# Autodesk Inventor assembly: bodyAssembly
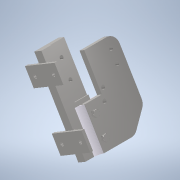
[picture p0: Inventor's stored thumbnail of the model, 180x180]
Saved by Autodesk Inventor 2020.3 (Build 243373000, 373)
## iProperties
Created: 2021-06-21
Part Number: bodyAssembly
Document SubType Name: Weldment
Designer: 0x6f736f646f
Weld Material: Welded Aluminum-6061
Author: 0x6f736f646f
## Documents named in this file (7)
- C:\Users\Public\D\Desktop\Trash\Manufacturing-Technology-1-Project\bodyAssembly.iam
- C:\Users\Public\D\Desktop\Trash\Manufacturing-Technology-1-Project\bodybottompart.ipt
- C:\Users\Public\D\Desktop\Trash\Manufacturing-Technology-1-Project\bodystandoff.ipt
- C:\Users\Public\D\Desktop\Trash\Manufacturing-Technology-1-Project\bodytoppart.ipt
- C:\Users\0x6f736f646f\OneDrive\Documents\Inventor\Content Center Files\R2020\en-US\BS EN ISO 8765\BS EN ISO 8765 - M10 x 1 x 50BS EN.ipt
- C:\Users\0x6f736f646f\OneDrive\Documents\Inventor\Content Center Files\R2020\en-US\AS 1112 (2)\AS 1112 - M10  Type 5.ipt
- C:\Users\0x6f736f646f\OneDrive\Documents\Inventor\Content Center Files\R2020\en-US\AS 1237 (2.1)\AS 1237 - 10.ipt
## Components (10 placed, 6 different names)
1. bodybottompart:1 — Mate:1, Mate:2, Mate:3, Mate:4, Mate:5, Mate:6, Mate:17, Mate:18
2. bodystandoff:1 — Mate:3, Mate:4
3. bodytoppart:1 — Mate:5, Mate:6, Mate:11, Mate:12, Mate:13, Mate:14
4. bodystandoff:2 — Mate:1, Mate:2
5. BS EN ISO 8765 - Metric M10 x 1 x 50:1 — Mate:7, Mate:8, Mate:11, Mate:15
6. BS EN ISO 8765 - Metric M10 x 1 x 50:2 — Mate:9, Mate:10, Mate:12, Mate:16
7. AS 1112 (2) - Metric M10  Type 5:1 — Mate:16, Mate:18
8. AS 1112 (2) - Metric M10  Type 5:2 — Mate:15, Mate:17
9. AS 1237 (2.1) 10:1 — Mate:7, Mate:8, Mate:13
10. AS 1237 (2.1) 10:2 — Mate:9, Mate:10, Mate:14
## Relationships (18: Mate 18)
- Mate:1: bodybottompart:1 ↔ bodystandoff:2
- Mate:2: bodybottompart:1 ↔ bodystandoff:2
- Mate:3: bodybottompart:1 ↔ bodystandoff:1
- Mate:4: bodybottompart:1 ↔ bodystandoff:1
- Mate:5: bodybottompart:1 ↔ bodytoppart:1
- Mate:6: bodybottompart:1 ↔ bodytoppart:1
- Mate:7: BS EN ISO 8765 - Metric M10 x 1 x 50:1 ↔ AS 1237 (2.1) 10:1
- Mate:8: BS EN ISO 8765 - Metric M10 x 1 x 50:1 ↔ AS 1237 (2.1) 10:1
- Mate:9: BS EN ISO 8765 - Metric M10 x 1 x 50:2 ↔ AS 1237 (2.1) 10:2
- Mate:10: BS EN ISO 8765 - Metric M10 x 1 x 50:2 ↔ AS 1237 (2.1) 10:2
- Mate:11: bodytoppart:1 ↔ BS EN ISO 8765 - Metric M10 x 1 x 50:1
- Mate:12: bodytoppart:1 ↔ BS EN ISO 8765 - Metric M10 x 1 x 50:2
- Mate:13: bodytoppart:1 ↔ AS 1237 (2.1) 10:1
- Mate:14: bodytoppart:1 ↔ AS 1237 (2.1) 10:2
- Mate:15: BS EN ISO 8765 - Metric M10 x 1 x 50:1 ↔ AS 1112 (2) - Metric M10  Type 5:2
- Mate:16: BS EN ISO 8765 - Metric M10 x 1 x 50:2 ↔ AS 1112 (2) - Metric M10  Type 5:1
- Mate:17: bodybottompart:1 ↔ AS 1112 (2) - Metric M10  Type 5:2
- Mate:18: bodybottompart:1 ↔ AS 1112 (2) - Metric M10  Type 5:1
